# Autodesk Inventor assembly: ASSEMBLY_Balcony_Mounting_Clamp
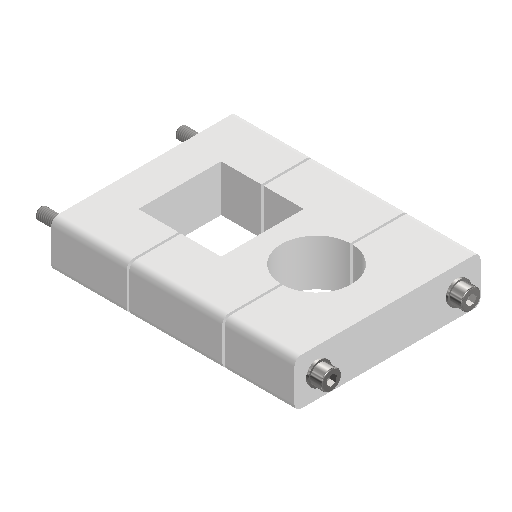
[picture p0: Inventor's stored thumbnail of the model, 512x512]
Saved by Autodesk Inventor 2026.1 (Build 301233000, 233)
## iProperties
Created: 2025-06-22
Part Number: ASSEMBLY_Balcony_Mounting_Clamp
Document SubType Name: Assembly
Designer: User
Author: User
## Documents named in this file (7)
- C:\Users\Andrzej\OneDrive\_DRIVE_SYNCH_FILES\__ BYTECHLAB PROJECTS\RF - Mostly 3D Printed Discone Antenna\MCAD\15_DISCONE_V4\ASSEMBLY_MAIN_REVA\ASSEMBLY_Balcony_Mounting_Clamp.iam
- C:\Users\Andrzej\OneDrive\_DRIVE_SYNCH_FILES\__ BYTECHLAB PROJECTS\RF - Mostly 3D Printed Discone Antenna\MCAD\15_DISCONE_V4\ASSEMBLY_MAIN_REVA\3DP_ASA_Balcony_Mounting_Clamp_Back.ipt
- C:\Users\Andrzej\OneDrive\_DRIVE_SYNCH_FILES\__ BYTECHLAB PROJECTS\RF - Mostly 3D Printed Discone Antenna\MCAD\15_DISCONE_V4\ASSEMBLY_MAIN_REVA\3DP_ASA_Balcony_Mounting_Clamp_Front.ipt
- C:\Users\Andrzej\OneDrive\_DRIVE_SYNCH_FILES\__ BYTECHLAB PROJECTS\RF - Mostly 3D Printed Discone Antenna\MCAD\15_DISCONE_V4\ASSEMBLY_MAIN_REVA\3DP_ASA_Balcony_Mounting_Clamp_Mid.ipt
- C:\Users\Andrzej\OneDrive\_DRIVE_SYNCH_FILES\__ BYTECHLAB PROJECTS\RF - Mostly 3D Printed Discone Antenna\MCAD\15_DISCONE_V4\__COTS_PARTS\COTS_GENERIC_DIN 912 - M5x120.ipt
- C:\Users\Andrzej\OneDrive\_DRIVE_SYNCH_FILES\__ BYTECHLAB PROJECTS\RF - Mostly 3D Printed Discone Antenna\MCAD\15_DISCONE_V4\__CONTENT_CENTER_PARTS\en-US\DIN 125-1  A\DIN 125 - A 5,3.ipt
- C:\Users\Andrzej\OneDrive\_DRIVE_SYNCH_FILES\__ BYTECHLAB PROJECTS\RF - Mostly 3D Printed Discone Antenna\MCAD\15_DISCONE_V4\__CONTENT_CENTER_PARTS\en-US\DIN 934\DIN 934 - M5 x 0,8.ipt
## Components (11 placed, 6 different names)
1. 3DP_ASA_Balcony_Mounting_Clamp_Back:1 — Mate:1, Flush:1, Flush:2, Insert:3, Insert:4
2. 3DP_ASA_Balcony_Mounting_Clamp_Front:1 — Mate:2, Flush:3, Flush:4, Mate:3, Mate:4, Insert:1, Insert:2
3. 3DP_ASA_Balcony_Mounting_Clamp_Mid:1 — Mate:1, Flush:1, Flush:2, Mate:2, Flush:3, Flush:4
4. COTS_GENERIC_DIN 912 - M5x120:1 — Mate:3, Mate:6
5. COTS_GENERIC_DIN 912 - M5x120:2 — Mate:4, Mate:5
6. DIN 125-1 A A 5,3:1 — Insert:1, Mate:5
7. DIN 125-1 A A 5,3:2 — Insert:2, Mate:6
8. DIN 125-1 A A 5,3:3 — Insert:3, Insert:5
9. DIN 125-1 A A 5,3:4 — Insert:4, Insert:6
10. DIN 934 - replaced by DIN EN 24032/28673/28674 M5:1 — Insert:5
11. DIN 934 - replaced by DIN EN 24032/28673/28674 M5:2 — Insert:6
## Relationships (16: Mate 6, Insert 6, Flush 4)
- Mate:1 (1 mm): 3DP_ASA_Balcony_Mounting_Clamp_Back:1 ↔ 3DP_ASA_Balcony_Mounting_Clamp_Mid:1
- Flush:1: 3DP_ASA_Balcony_Mounting_Clamp_Back:1 ↔ 3DP_ASA_Balcony_Mounting_Clamp_Mid:1
- Flush:2: 3DP_ASA_Balcony_Mounting_Clamp_Back:1 ↔ 3DP_ASA_Balcony_Mounting_Clamp_Mid:1
- Mate:2 (1 mm): 3DP_ASA_Balcony_Mounting_Clamp_Front:1 ↔ 3DP_ASA_Balcony_Mounting_Clamp_Mid:1
- Flush:3: 3DP_ASA_Balcony_Mounting_Clamp_Front:1 ↔ 3DP_ASA_Balcony_Mounting_Clamp_Mid:1
- Flush:4: 3DP_ASA_Balcony_Mounting_Clamp_Front:1 ↔ 3DP_ASA_Balcony_Mounting_Clamp_Mid:1
- Mate:3: 3DP_ASA_Balcony_Mounting_Clamp_Front:1 ↔ COTS_GENERIC_DIN 912 - M5x120:1
- Mate:4: 3DP_ASA_Balcony_Mounting_Clamp_Front:1 ↔ COTS_GENERIC_DIN 912 - M5x120:2
- Insert:1: 3DP_ASA_Balcony_Mounting_Clamp_Front:1 ↔ DIN 125-1 A A 5,3:1
- Insert:2: 3DP_ASA_Balcony_Mounting_Clamp_Front:1 ↔ DIN 125-1 A A 5,3:2
- Insert:3: 3DP_ASA_Balcony_Mounting_Clamp_Back:1 ↔ DIN 125-1 A A 5,3:3
- Insert:4: 3DP_ASA_Balcony_Mounting_Clamp_Back:1 ↔ DIN 125-1 A A 5,3:4
- Mate:5: COTS_GENERIC_DIN 912 - M5x120:2 ↔ DIN 125-1 A A 5,3:1
- Mate:6: COTS_GENERIC_DIN 912 - M5x120:1 ↔ DIN 125-1 A A 5,3:2
- Insert:5: DIN 125-1 A A 5,3:3 ↔ DIN 934 - replaced by DIN EN 24032/28673/28674 M5:1
- Insert:6: DIN 125-1 A A 5,3:4 ↔ DIN 934 - replaced by DIN EN 24032/28673/28674 M5:2
